# Autodesk Inventor assembly: Máy Nén Khí
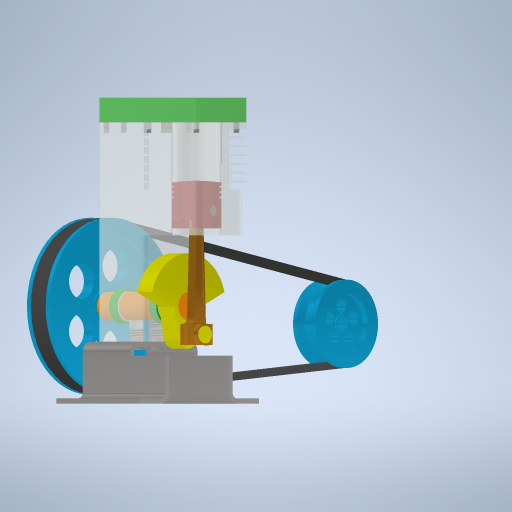
[picture p0: Inventor's stored thumbnail of the model, 512x512]
Saved by Autodesk Inventor 2023 (Build 270158000, 158)
## iProperties
Created: 2023-10-08
Part Number: Máy Nén Khí
Document SubType Name: Assembly
Designer: huy20
Author: huy20
## Documents named in this file (18)
- C:\Users\huy20\OneDrive\Máy tính\Inventor\TK Cơ cấu cơ khi\Máy Nén Khí.iam
- C:\Users\huy20\OneDrive\Máy tính\Inventor\TK Cơ cấu cơ khi\Chi tiết\Máy Nén Khí\Giá đỡ.ipt
- C:\Users\huy20\OneDrive\Máy tính\Inventor\TK Cơ cấu cơ khi\Chi tiết\Máy Nén Khí\Hộp Piston .ipt
- C:\Users\huy20\OneDrive\Máy tính\Inventor\TK Cơ cấu cơ khi\Chi tiết\Máy Nén Khí\Piston.ipt
- C:\Users\huy20\OneDrive\Máy tính\Inventor\TK Cơ cấu cơ khi\Chi tiết\Máy Nén Khí\Piston Pin.ipt
- C:\Users\huy20\OneDrive\Máy tính\Inventor\TK Cơ cấu cơ khi\Chi tiết\Máy Nén Khí\Thanh Truyen 1.ipt
- C:\Users\huy20\OneDrive\Máy tính\Inventor\TK Cơ cấu cơ khi\Chi tiết\Máy Nén Khí\Thanh Truyen.ipt
- C:\Users\huy20\OneDrive\Máy tính\Inventor\TK Cơ cấu cơ khi\Chi tiết\Máy Nén Khí\Crank.ipt
- C:\Users\huy20\OneDrive\Máy tính\Inventor\TK Cơ cấu cơ khi\Chi tiết\Máy Nén Khí\Trục.ipt
- C:\Users\huy20\OneDrive\Máy tính\Inventor\TK Cơ cấu cơ khi\Chi tiết\Máy Nén Khí\Pulley lớn.ipt
- C:\Users\huy20\OneDrive\Máy tính\Inventor\TK Cơ cấu cơ khi\Chi tiết\Máy Nén Khí\Pulley nhỏ.ipt
- C:\Users\huy20\OneDrive\Máy tính\Inventor\TK Cơ cấu cơ khi\Chi tiết\Máy Nén Khí\Nắp hộp piston.ipt
- C:\Users\huy20\OneDrive\Máy tính\Inventor\TK Cơ cấu cơ khi\Chi tiết\Máy Nén Khí\Dây đai.ipt
- C:\Users\huy20\OneDrive\Máy tính\Inventor\TK Cơ cấu cơ khi\Chi tiết\Máy Nén Khí\Vòng Bi.iam
- C:\Users\huy20\OneDrive\Documents\Inventor\Content Center Files\R2023\en-US\ANSI B18.3.1M(1)\ANSI B18.3.1M - M1.6x0.35 x 8(2).ipt
- C:\Users\huy20\OneDrive\Máy tính\Inventor\TK Cơ cấu cơ khi\Chi tiết\Máy Nén Khí\Trục Pin.ipt
- C:\Users\huy20\OneDrive\Documents\Inventor\Content Center Files\R2023\en-US\ISO 7436(4)\ISO 7436 - M1.6 x 6 - DIN EN.ipt
- C:\Users\huy20\OneDrive\Documents\Inventor\Content Center Files\R2023\en-US\DIN 920\DIN 920 - M4 x 4.ipt
## Components (29 placed, 17 different names)
1. Giá đỡ:1 — Mate:1, Flush:1, Flush:2, Mate:2, Mate:3, Mate:4
2. Hộp Piston :1 — Mate:2, Mate:3, Mate:4, Mate:5, Mate:12, Mate:20, Mate:25, Flush:6, Mate:29, Flush:9, Mate:30, Flush:10, Mate:57, Mate:58, Mate:59, Mate:60
3. Piston:1 — Mate:5, Mate:7, Mate:11, Mate:17
4. Piston Pin:1 — Mate:7, Mate:10, Mate:17
5. Thanh Truyen 1:1 — Mate:8, Mate:9, Flush:3, Mate:55, Mate:56
6. Thanh Truyen:1 — Mate:8, Mate:9, Flush:3, Mate:10, Mate:11, Mate:15, Mate:16, Chuyen Dong
7. Crank:1 — Mate:13, Flush:4, Mate:14, Mate:15, Mate:16, Angle:1, Mate:53
8. Trục:1 — Mate:12, Mate:13, Flush:4, Mate:14, Mate:18, Mate:19, Flush:5, Angle:1, Angle:5, Flush:11, Mate:54, Flush:13
9. Pulley lớn:1 — Mate:18, Mate:19, Flush:5, Chuyen Dong, Mate:26, Flush:7, Flush:8, Angle:3, Flush:12
10. Pulley nhỏ:1 — Mate:26, Mate:28, Angle:3
11. Nắp hộp piston:1 — Mate:20, Mate:25, Flush:6, Mate:35, Mate:36, Mate:37, Mate:38, Mate:39, Mate:40, Mate:41, Mate:42, Mate:43, Mate:44, Mate:45, Mate:46, Mate:47, Mate:48, Mate:49, Mate:50, Mate:51, Mate:52
12. Dây đai:1 — Flush:8, Mate:28
13. Vòng Bi:1 [sub-assembly] — Mate:30, Flush:10, Angle:4
14. Vòng Bi:2 [sub-assembly] — Mate:29, Flush:9, Angle:4, Angle:5
15. Broached Socket Head Cap Screw - Metric M1.6x0.35 x 8:1 — Mate:35, Mate:36
16. Broached Socket Head Cap Screw - Metric M1.6x0.35 x 8:2 — Mate:37, Mate:38
17. Broached Socket Head Cap Screw - Metric M1.6x0.35 x 8:3 — Mate:39, Mate:40
18. Broached Socket Head Cap Screw - Metric M1.6x0.35 x 8:4 — Mate:41, Mate:42
19. Broached Socket Head Cap Screw - Metric M1.6x0.35 x 8:5 — Mate:43, Mate:44
20. Broached Socket Head Cap Screw - Metric M1.6x0.35 x 8:6 — Mate:45, Mate:46
21. Broached Socket Head Cap Screw - Metric M1.6x0.35 x 8:7 — Mate:47, Mate:48
22. Broached Socket Head Cap Screw - Metric M1.6x0.35 x 8:8 — Mate:49, Mate:50
23. Broached Socket Head Cap Screw - Metric M1.6x0.35 x 8:9 — Mate:51, Mate:52
24. Trục Pin:1 — Mate:54, Flush:12, Flush:13
25. Trục Pin:2 — Mate:53, Flush:11
26. DIN EN 27436 M1.6 x 6:1 — Mate:55
27. DIN EN 27436 M1.6 x 6:2 — Mate:56
28. DIN 920 M4 x 4:1 — Mate:57, Mate:58
29. DIN 920 M4 x 4:2 — Mate:59, Mate:60
## Relationships (68: Mate 50, Flush 13, Angle 5)
- Mate:1: Giá đỡ:1
- Flush:1: Giá đỡ:1
- Flush:2: Giá đỡ:1
- Mate:2: Giá đỡ:1 ↔ Hộp Piston :1
- Mate:3: Giá đỡ:1 ↔ Hộp Piston :1
- Mate:4: Giá đỡ:1 ↔ Hộp Piston :1
- Mate:5: Hộp Piston :1 ↔ Piston:1
- Mate:7: Piston:1 ↔ Piston Pin:1
- Mate:8: Thanh Truyen 1:1 ↔ Thanh Truyen:1
- Mate:9: Thanh Truyen 1:1 ↔ Thanh Truyen:1
- Flush:3: Thanh Truyen 1:1 ↔ Thanh Truyen:1
- Mate:10: Piston Pin:1 ↔ Thanh Truyen:1
- Mate:11: Piston:1 ↔ Thanh Truyen:1
- Mate:12: Hộp Piston :1 ↔ Trục:1
- Mate:13: Crank:1 ↔ Trục:1
- Flush:4: Crank:1 ↔ Trục:1
- Mate:14: Crank:1 ↔ Trục:1
- Mate:15: Thanh Truyen:1 ↔ Crank:1
- Mate:16: Thanh Truyen:1 ↔ Crank:1
- Mate:17: Piston:1 ↔ Piston Pin:1
- Mate:18: Trục:1 ↔ Pulley lớn:1
- Mate:19: Trục:1 ↔ Pulley lớn:1
- Flush:5: Trục:1 ↔ Pulley lớn:1
- Angle:1 (0 deg): Crank:1 ↔ Trục:1
- Chuyen Dong [Angle] (0 deg): Thanh Truyen:1 ↔ Pulley lớn:1
- Mate:20: Hộp Piston :1 ↔ Nắp hộp piston:1
- Mate:25: Hộp Piston :1 ↔ Nắp hộp piston:1
- Flush:6: Hộp Piston :1 ↔ Nắp hộp piston:1
- Mate:26: Pulley lớn:1 ↔ Pulley nhỏ:1
- Flush:7: Pulley lớn:1
- Flush:8: Pulley lớn:1 ↔ Dây đai:1
- Mate:28: Pulley nhỏ:1 ↔ Dây đai:1
- Angle:3 (0 deg): Pulley lớn:1 ↔ Pulley nhỏ:1
- Mate:29: Hộp Piston :1 ↔ Vòng Bi:2
- Flush:9: Hộp Piston :1 ↔ Vòng Bi:2
- Mate:30: Hộp Piston :1 ↔ Vòng Bi:1
- Flush:10: Hộp Piston :1 ↔ Vòng Bi:1
- Angle:4 (0 deg): Vòng Bi:1 ↔ Vòng Bi:2
- Angle:5 (0 deg): Trục:1 ↔ Vòng Bi:2
- Mate:35: Nắp hộp piston:1 ↔ Broached Socket Head Cap Screw - Metric M1.6x0.35 x 8:1
- Mate:36: Nắp hộp piston:1 ↔ Broached Socket Head Cap Screw - Metric M1.6x0.35 x 8:1
- Mate:37: Nắp hộp piston:1 ↔ Broached Socket Head Cap Screw - Metric M1.6x0.35 x 8:2
- Mate:38: Nắp hộp piston:1 ↔ Broached Socket Head Cap Screw - Metric M1.6x0.35 x 8:2
- Mate:39: Nắp hộp piston:1 ↔ Broached Socket Head Cap Screw - Metric M1.6x0.35 x 8:3
- Mate:40: Nắp hộp piston:1 ↔ Broached Socket Head Cap Screw - Metric M1.6x0.35 x 8:3
- Mate:41: Nắp hộp piston:1 ↔ Broached Socket Head Cap Screw - Metric M1.6x0.35 x 8:4
- Mate:42: Nắp hộp piston:1 ↔ Broached Socket Head Cap Screw - Metric M1.6x0.35 x 8:4
- Mate:43: Nắp hộp piston:1 ↔ Broached Socket Head Cap Screw - Metric M1.6x0.35 x 8:5
- Mate:44: Nắp hộp piston:1 ↔ Broached Socket Head Cap Screw - Metric M1.6x0.35 x 8:5
- Mate:45: Nắp hộp piston:1 ↔ Broached Socket Head Cap Screw - Metric M1.6x0.35 x 8:6
- Mate:46: Nắp hộp piston:1 ↔ Broached Socket Head Cap Screw - Metric M1.6x0.35 x 8:6
- Mate:47: Nắp hộp piston:1 ↔ Broached Socket Head Cap Screw - Metric M1.6x0.35 x 8:7
- Mate:48: Nắp hộp piston:1 ↔ Broached Socket Head Cap Screw - Metric M1.6x0.35 x 8:7
- Mate:49: Nắp hộp piston:1 ↔ Broached Socket Head Cap Screw - Metric M1.6x0.35 x 8:8
- Mate:50: Nắp hộp piston:1 ↔ Broached Socket Head Cap Screw - Metric M1.6x0.35 x 8:8
- Mate:51: Nắp hộp piston:1 ↔ Broached Socket Head Cap Screw - Metric M1.6x0.35 x 8:9
- Mate:52: Nắp hộp piston:1 ↔ Broached Socket Head Cap Screw - Metric M1.6x0.35 x 8:9
- Mate:53: Crank:1 ↔ Trục Pin:2
- Flush:11: Trục:1 ↔ Trục Pin:2
- Mate:54: Trục:1 ↔ Trục Pin:1
- Flush:12: Pulley lớn:1 ↔ Trục Pin:1
- Flush:13: Trục:1 ↔ Trục Pin:1
- Mate:55: Thanh Truyen 1:1 ↔ DIN EN 27436 M1.6 x 6:1
- Mate:56: Thanh Truyen 1:1 ↔ DIN EN 27436 M1.6 x 6:2
- Mate:57: Hộp Piston :1 ↔ DIN 920 M4 x 4:1
- Mate:58: Hộp Piston :1 ↔ DIN 920 M4 x 4:1
- Mate:59: Hộp Piston :1 ↔ DIN 920 M4 x 4:2
- Mate:60: Hộp Piston :1 ↔ DIN 920 M4 x 4:2
